# Autodesk Inventor assembly: The Bump
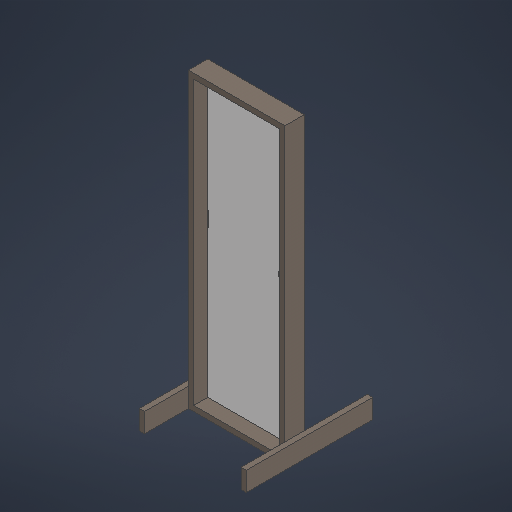
[picture p0: Inventor's stored thumbnail of the model, 512x512]
Saved by Autodesk Inventor 2025.1 (Build 291241020, 241B)
## iProperties
Created: 2026-03-06
Part Number: The Bump
Document SubType Name: Assembly
Designer: brand
Author: brand
## Documents named in this file (6)
- C:\Users\brand\OneDrive\Documents\Dash\Desktop\The Bump.iam
- C:\Users\brand\Downloads\1518A15_Single Door\1518A15_Single Door\1518A15_Single Door.ipt
- C:\Users\brand\DoorFrame.ipt
- C:\Users\brand\Downloads\1494A43_Mortise-Mount Entry Door Template Hinge\1494A43_Mortise-Mount Entry Door Template Hinge\1494A43_Mortise-Mount Entry Door Template Hinge.ipt
- C:\Users\brand\Downloads\1494A43_Mortise-Mount Entry Door Template Hinge\1494A43_Mortise-Mount Entry Door Template Hinge\Hinge1.ipt
- C:\Users\brand\OneDrive\Documents\Dash\Desktop\DoorFrameBase.ipt
## Components (6 placed, 5 different names)
1. 1518A15_Single Door:1 — Flush:1, Flush:2, Mate:1
2. DoorFrame:1 — Flush:1, Flush:2, Mate:2, Angle:1, Flush:3, Flush:4, Flush:5, Mate:3, Flush:6
3. 1494A43_Mortise-Mount Entry Door Template Hinge:2 — Mate:1, Mate:2, Angle:1, Flush:3, Insert:1
4. Hinge1:1 — Insert:1
5. DoorFrameBase:1 — Flush:4, Flush:5, Flush:7
6. DoorFrameBase:2 — Mate:3, Flush:6, Flush:7
## Relationships (12: Flush 7, Mate 3, Angle 1, Insert 1)
- Flush:1: 1518A15_Single Door:1 ↔ DoorFrame:1
- Flush:2: 1518A15_Single Door:1 ↔ DoorFrame:1
- Mate:1: 1518A15_Single Door:1 ↔ 1494A43_Mortise-Mount Entry Door Template Hinge:2
- Mate:2: DoorFrame:1 ↔ 1494A43_Mortise-Mount Entry Door Template Hinge:2
- Angle:1 (0 deg): DoorFrame:1 ↔ 1494A43_Mortise-Mount Entry Door Template Hinge:2
- Flush:3: DoorFrame:1 ↔ 1494A43_Mortise-Mount Entry Door Template Hinge:2
- Insert:1: 1494A43_Mortise-Mount Entry Door Template Hinge:2 ↔ Hinge1:1
- Flush:4: DoorFrame:1 ↔ DoorFrameBase:1
- Flush:5: DoorFrame:1 ↔ DoorFrameBase:1
- Mate:3: DoorFrame:1 ↔ DoorFrameBase:2
- Flush:6: DoorFrame:1 ↔ DoorFrameBase:2
- Flush:7: DoorFrameBase:1 ↔ DoorFrameBase:2
